# Autodesk Inventor assembly: Hip-40x
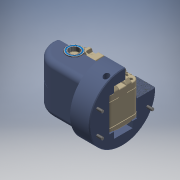
[picture p0: Inventor's stored thumbnail of the model, 180x180]
Saved by Autodesk Inventor 2018 (Build 220112000, 112)
## iProperties
Created: 2017-10-09
Part Number: Hip-40x
Material: Generisch
Document SubType Name: Assembly
Designer: JochenAlt
Author: JochenAlt
## Documents named in this file (6)
- D:\Projects\Manfred\design\cad\Inventor\Hip-40x.iam
- D:\Projects\Manfred\design\cad\Inventor\Herkulex DRS-010x\HerkuleX DRS-0101.iam
- D:\Projects\Manfred\design\cad\Inventor\Rillenkugellager 11x7x3 inafag smr117.ipt
- D:\Projects\Manfred\design\cad\Inventor\Hip-40x.ipt
- C:\Users\JochenAlt\Documents\Inventor\Content Center Files\R2018\de-DE\ISO 4762(1)\DIN EN ISO 4762 - M2 x 3.ipt
- C:\Users\JochenAlt\Documents\Inventor\Content Center Files\R2018\de-DE\ISO 4762(1)\DIN EN ISO 4762 - M2 x 8.ipt
## Components (11 placed, 5 different names)
1. HerkuleX DRS-0101:1 [sub-assembly] — Passend:1, Passend:2, Passend:3, Passend:4, Passend:5
2. Rillenkugellager 11x7x3 inafag smr117:1 — Passend:1, Passend:2
3. Hip-40x:1 — Passend:3, Passend:4, Passend:5, Einfügen:1, Einfügen:2, Einfügen:3, Einfügen:4, Einfügen:5, Einfügen:6, Einfügen:7, Einfügen:8
4. DIN EN ISO 4762 M2 x 3:1 — Einfügen:1
5. DIN EN ISO 4762 M2 x 3:2 — Einfügen:2
6. DIN EN ISO 4762 M2 x 3:3 — Einfügen:3
7. DIN EN ISO 4762 M2 x 3:4 — Einfügen:4
8. DIN EN ISO 4762 M2 x 8:1 — Einfügen:5
9. DIN EN ISO 4762 M2 x 8:2 — Einfügen:6
10. DIN EN ISO 4762 M2 x 8:3 — Einfügen:7
11. DIN EN ISO 4762 M2 x 8:4 — Einfügen:8
## Relationships (13: Insert 8, Mate 5)
- Passend:1 [Mate]: HerkuleX DRS-0101:1 ↔ Rillenkugellager 11x7x3 inafag smr117:1
- Passend:2 [Mate] (0.2 mm): HerkuleX DRS-0101:1 ↔ Rillenkugellager 11x7x3 inafag smr117:1
- Passend:3 [Mate]: HerkuleX DRS-0101:1 ↔ Hip-40x:1
- Passend:4 [Mate]: HerkuleX DRS-0101:1 ↔ Hip-40x:1
- Passend:5 [Mate] (0.1 mm): HerkuleX DRS-0101:1 ↔ Hip-40x:1
- Einfügen:1 [Insert]: Hip-40x:1 ↔ DIN EN ISO 4762 M2 x 3:1
- Einfügen:2 [Insert]: Hip-40x:1 ↔ DIN EN ISO 4762 M2 x 3:2
- Einfügen:3 [Insert]: Hip-40x:1 ↔ DIN EN ISO 4762 M2 x 3:3
- Einfügen:4 [Insert]: Hip-40x:1 ↔ DIN EN ISO 4762 M2 x 3:4
- Einfügen:5 [Insert]: Hip-40x:1 ↔ DIN EN ISO 4762 M2 x 8:1
- Einfügen:6 [Insert]: Hip-40x:1 ↔ DIN EN ISO 4762 M2 x 8:2
- Einfügen:7 [Insert]: Hip-40x:1 ↔ DIN EN ISO 4762 M2 x 8:3
- Einfügen:8 [Insert]: Hip-40x:1 ↔ DIN EN ISO 4762 M2 x 8:4
